# Autodesk Inventor assembly: SCARA
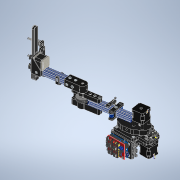
[picture p0: Inventor's stored thumbnail of the model, 180x180]
Saved by Autodesk Inventor 2022 (Build 260153000, 153)
## iProperties
Created: 2022-03-02
Part Number: SCARA
Document SubType Name: Assembly
Designer: JK
Author: JK
## Documents named in this file (5)
- C:\Users\JK\Documents\Inventor\ScaraNema\SCARA-3DP\Parts\SCARA.iam
- C:\Users\JK\Documents\Inventor\ScaraNema\SCARA-3DP\Parts\Shoulder\Shoulder base.iam
- C:\Users\JK\Documents\Inventor\ScaraNema\SCARA-3DP\Parts\Forearm\Forearm assembly.iam
- C:\Users\JK\Documents\Inventor\ScaraNema\SCARA-3DP\Parts\Arm\Arm Assembly.iam
- C:\Users\JK\Documents\Inventor\ScaraNema\SCARA-3DP\Parts\Electronics\Electronics.iam
## Components (4 placed, 4 different names)
1. Shoulder base:1 [sub-assembly] — Coincidencia:2, Coincidencia:3, Coincidencia:4, Nivelación:2, Nivelación:3
2. Forearm assembly:1 [sub-assembly] — Coincidencia:1, Coincidencia:5
3. Arm Assembly:1 [sub-assembly] — Coincidencia:1, Coincidencia:2, Coincidencia:3, Coincidencia:5
4. Electronics:1 [sub-assembly] — Coincidencia:4, Nivelación:2, Nivelación:3
## Relationships (7: Mate 5, Flush 2)
- Coincidencia:1 [Mate]: Forearm assembly:1 ↔ Arm Assembly:1
- Coincidencia:2 [Mate]: Shoulder base:1 ↔ Arm Assembly:1
- Coincidencia:3 [Mate]: Shoulder base:1 ↔ Arm Assembly:1
- Coincidencia:4 [Mate]: Shoulder base:1 ↔ Electronics:1
- Nivelación:2 [Flush]: Shoulder base:1 ↔ Electronics:1
- Nivelación:3 [Flush]: Shoulder base:1 ↔ Electronics:1
- Coincidencia:5 [Mate]: Forearm assembly:1 ↔ Arm Assembly:1
